# Autodesk Inventor assembly: Washing Machine Mock Up Assembly
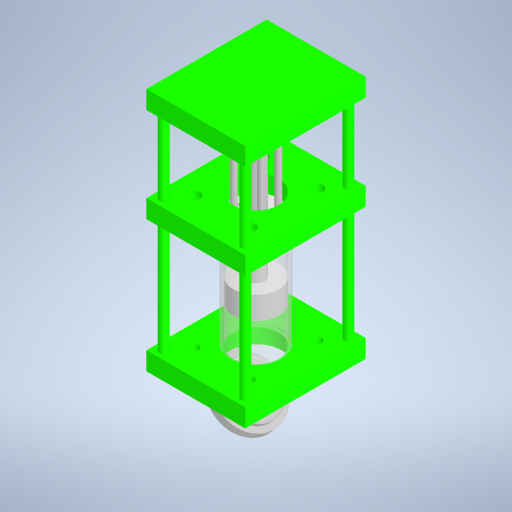
[picture p0: Inventor's stored thumbnail of the model, 512x512]
Saved by Autodesk Inventor 2023 (Build 270158000, 158)
## iProperties
Created: 2022-04-19
Part Number: Washing Machine Mock Up Assembly
Document SubType Name: Assembly
Designer: tgr41
Author: tgr41
## Documents named in this file (9)
- C:\Users\tommy\Documents\Repositories\Microgravity-Press-Washing-Machine\Old Resources\Mock Up Design\Washing Machine Mock Up Assembly.iam
- C:\Users\tommy\Documents\Repositories\Microgravity-Press-Washing-Machine\Old Resources\Mock Up Design\Parts\Wash_Base_Bottom.ipt
- C:\Users\tommy\Documents\Repositories\Microgravity-Press-Washing-Machine\Old Resources\Mock Up Design\Parts\Access Hatch.ipt
- C:\Users\tommy\Documents\Repositories\Microgravity-Press-Washing-Machine\Old Resources\Mock Up Design\Parts\Acting Piston.ipt
- C:\Users\tommy\Documents\Repositories\Microgravity-Press-Washing-Machine\Old Resources\Mock Up Design\Parts\Chamber Top.ipt
- C:\Users\tommy\Documents\Repositories\Microgravity-Press-Washing-Machine\Old Resources\Mock Up Design\Parts\Frame Rod.ipt
- C:\Users\tommy\Documents\Repositories\Microgravity-Press-Washing-Machine\Old Resources\Mock Up Design\Parts\Wash_Base_Middle.ipt
- C:\Users\tommy\Documents\Repositories\Microgravity-Press-Washing-Machine\Old Resources\Mock Up Design\Parts\Wash_Chamber_Pipe.ipt
- C:\Users\tommy\Documents\Repositories\Microgravity-Press-Washing-Machine\Old Resources\Mock Up Design\Parts\Wash_Base_Top.ipt
## Components (11 placed, 8 different names)
1. Wash_Base_Bottom:1 — Mate:1, Mate:2, Mate:3, Mate:4, Angle:1, Mate:5, Mate:6, Mate:7, Mate:8, Flush:1, Flush:2, Flush:3, Flush:4
2. Access Hatch:1 — Mate:3, Mate:4, Angle:1
3. Acting Piston:1 — Mate:13, Mate:14, Flush:6, Mate:15
4. Chamber Top:1 — Mate:14, Flush:5, Mate:15
5. Wash_Base_Middle:1 — Mate:10, Mate:11, Mate:12, Mate:18
6. Wash_Chamber_Pipe:1 — Mate:1, Mate:2, Mate:10, Mate:13, Flush:5, Flush:6, Mate:18
7. Frame Rod:2 — Mate:6, Flush:4, Mate:12
8. Frame Rod:3 — Mate:7, Flush:2, Mate:11, Mate:17
9. Frame Rod:4 — Mate:8, Flush:3
10. Frame Rod:5 — Mate:5, Flush:1, Flush:7, Mate:16
11. Wash_Base_Top:1 — Flush:7, Mate:16, Mate:17
## Relationships (25: Mate 17, Flush 7, Angle 1)
- Mate:1: Wash_Base_Bottom:1 ↔ Wash_Chamber_Pipe:1
- Mate:2: Wash_Base_Bottom:1 ↔ Wash_Chamber_Pipe:1
- Mate:3: Wash_Base_Bottom:1 ↔ Access Hatch:1
- Mate:4: Wash_Base_Bottom:1 ↔ Access Hatch:1
- Angle:1 (0 deg): Wash_Base_Bottom:1 ↔ Access Hatch:1
- Mate:5: Wash_Base_Bottom:1 ↔ Frame Rod:5
- Mate:6: Wash_Base_Bottom:1 ↔ Frame Rod:2
- Mate:7: Wash_Base_Bottom:1 ↔ Frame Rod:3
- Mate:8: Wash_Base_Bottom:1 ↔ Frame Rod:4
- Flush:1: Wash_Base_Bottom:1 ↔ Frame Rod:5
- Flush:2: Wash_Base_Bottom:1 ↔ Frame Rod:3
- Flush:3: Wash_Base_Bottom:1 ↔ Frame Rod:4
- Flush:4: Wash_Base_Bottom:1 ↔ Frame Rod:2
- Mate:10: Wash_Base_Middle:1 ↔ Wash_Chamber_Pipe:1
- Mate:11: Wash_Base_Middle:1 ↔ Frame Rod:3
- Mate:12: Wash_Base_Middle:1 ↔ Frame Rod:2
- Mate:13: Acting Piston:1 ↔ Wash_Chamber_Pipe:1
- Mate:14: Acting Piston:1 ↔ Chamber Top:1
- Flush:5: Chamber Top:1 ↔ Wash_Chamber_Pipe:1
- Flush:6: Acting Piston:1 ↔ Wash_Chamber_Pipe:1
- Mate:15: Acting Piston:1 ↔ Chamber Top:1
- Flush:7: Frame Rod:5 ↔ Wash_Base_Top:1
- Mate:16: Frame Rod:5 ↔ Wash_Base_Top:1
- Mate:17: Frame Rod:3 ↔ Wash_Base_Top:1
- Mate:18: Wash_Base_Middle:1 ↔ Wash_Chamber_Pipe:1
